# Autodesk Inventor assembly: upper long wall
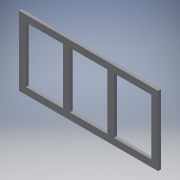
[picture p0: Inventor's stored thumbnail of the model, 180x180]
Saved by Autodesk Inventor 2017 (Build 210142000, 142)
## iProperties
Created: 2019-05-06
Part Number: upper long wall
Document SubType Name: Assembly
Designer: Roman
Author: Roman
## Documents named in this file (3)
- C:\Users\Roman\Documents\CAD\tegu rev2\upper walls\long wall\upper long wall.iam
- C:\Users\Roman\Documents\CAD\tegu rev2\upper walls\long wall\upper long wall h bar.ipt
- C:\Users\Roman\Documents\CAD\tegu rev2\upper walls\long wall\upper long wall v bar.ipt
## Components (6 placed, 2 different names)
1. upper long wall h bar:1 — Mate:1, Flush:1, Flush:2
2. upper long wall h bar:2 — Mate:2, Flush:3, Flush:4
3. upper long wall v bar:1 — Mate:1, Flush:1, Flush:2, Mate:2, Flush:3, Flush:4
4. upper long wall v bar:2
5. upper long wall v bar:3
6. upper long wall v bar:4
## Component patterns: (4 elements, first: upper long wall v bar:1)
## Relationships (6: Flush 4, Mate 2)
- Mate:1: upper long wall h bar:1 ↔ upper long wall v bar:1
- Flush:1: upper long wall h bar:1 ↔ upper long wall v bar:1
- Flush:2: upper long wall h bar:1 ↔ upper long wall v bar:1
- Mate:2: upper long wall h bar:2 ↔ upper long wall v bar:1
- Flush:3: upper long wall h bar:2 ↔ upper long wall v bar:1
- Flush:4: upper long wall h bar:2 ↔ upper long wall v bar:1
